# Autodesk Inventor assembly: CL5-100
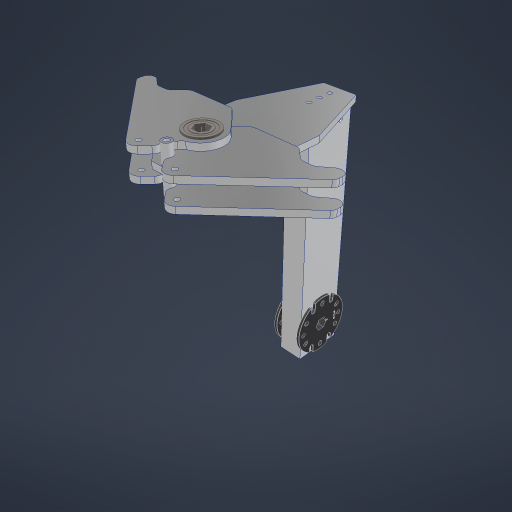
[picture p0: Inventor's stored thumbnail of the model, 512x512]
Saved by Autodesk Inventor 2023.4 (Build 274418000, 418)
## iProperties
Created: 2025-02-04
Part Number: CL5-100
Document SubType Name: Assembly
Designer: brand
Author: brand
## Documents named in this file (10)
- C:\Users\brand\OneDrive\Documents\GitHub\robotics 23\2025-ReefScape---CAD\Climber\CL5\CL5-100.iam
- C:\Users\brand\OneDrive\Documents\GitHub\robotics 23\2025-ReefScape---CAD\Field Items\Full Field\FE-2025\GE-25201.iam
- C:\Users\brand\OneDrive\Documents\GitHub\robotics 23\2025-ReefScape---CAD\Climber\CL4\02_Barb Assembly (1)\02_Barb Assembly (1).iam
- C:\Users\brand\OneDrive\Documents\GitHub\robotics 23\2025-ReefScape---CAD\COMMON PARTS\HUBS\WCP-1388.ipt
- C:\Users\brand\OneDrive\Documents\GitHub\robotics 23\2025-ReefScape---CAD\Climber\CL5\CL5-001.ipt
- C:\Users\brand\OneDrive\Documents\GitHub\robotics 23\2025-ReefScape---CAD\Elevator\EL2\EL2-005.ipt
- C:\Users\brand\OneDrive\Documents\GitHub\robotics 23\2025-ReefScape---CAD\Climber\CL5\CL5-002.ipt
- C:\Users\brand\OneDrive\Documents\GitHub\robotics 23\2025-ReefScape---CAD\Climber\CL5\CL5-003.ipt
- C:\Users\brand\OneDrive\Documents\GitHub\robotics 23\2025-ReefScape---CAD\Climber\CL5\CL5-004.ipt
- C:\Users\brand\OneDrive\Documents\GitHub\robotics 23\2025-ReefScape---CAD\COMMON PARTS\BEARINGS\0_500_Hex_ID_x_1_125_OD_x_0_313_WD_Flanged_Bearing_v2_217-3875.ipt
## Components (18 placed, 9 different names)
1. CL5-001:1 — Mate:7, Flush:6, Flush:7, Insert:2, Mate:14, Insert:3, Mate:15, Mate:16, Flush:9, Insert:11, Insert:12
2. GE-25201:1 [sub-assembly] — Mate:7
3. 02_Barb Assembly (1):1 [sub-assembly] — Flush:6, Flush:7
4. WCP-1388:1 — Insert:2, Mate:14
5. WCP-1388:2 — Insert:3, Mate:15
6. EL2-005:1 — Insert:11, Insert:12, Insert:13, Insert:14
7. CL5-002:1 — Mate:18, Mate:19, Mate:20, Mate:21, Flush:9, Insert:4, Insert:5, Insert:8, Insert:13, Insert:14
8. CL5-003:1 — Mate:18, Insert:9, Mate:26
9. CL5-004:1 — Insert:4, Mate:28, Mate:29
10. CL5-003:2 — Mate:21, Insert:7, Mate:28
11. CL5-003:4 — Mate:19, Insert:6, Mate:29
12. CL5-003:5 — Mate:20, Insert:10, Mate:27
13. CL5-004:2 — Insert:5, Mate:26, Mate:27
14. 0_500_Hex_ID_x_1_125_OD_x_0_313_WD_Flanged_Bearing_v2_217-3875:1 — Insert:8, Mate:22, Mate:24
15. 0_500_Hex_ID_x_1_125_OD_x_0_313_WD_Flanged_Bearing_v2_217-3875:2 — Insert:10, Mate:25
16. 0_500_Hex_ID_x_1_125_OD_x_0_313_WD_Flanged_Bearing_v2_217-3875:3 — Insert:9, Mate:24, Mate:25
17. 0_500_Hex_ID_x_1_125_OD_x_0_313_WD_Flanged_Bearing_v2_217-3875:4 — Insert:7, Mate:22, Mate:23
18. 0_500_Hex_ID_x_1_125_OD_x_0_313_WD_Flanged_Bearing_v2_217-3875:5 — Insert:6, Mate:23
## Relationships (32: Mate 16, Insert 13, Flush 3)
- Mate:7: CL5-001:1 ↔ GE-25201:1
- Flush:6: CL5-001:1 ↔ 02_Barb Assembly (1):1
- Flush:7: CL5-001:1 ↔ 02_Barb Assembly (1):1
- Insert:2: CL5-001:1 ↔ WCP-1388:1
- Mate:14: CL5-001:1 ↔ WCP-1388:1
- Insert:3: CL5-001:1 ↔ WCP-1388:2
- Mate:15: CL5-001:1 ↔ WCP-1388:2
- Mate:16: CL5-001:1
- Mate:18: CL5-002:1 ↔ CL5-003:1
- Mate:19: CL5-002:1 ↔ CL5-003:4
- Mate:20: CL5-002:1 ↔ CL5-003:5
- Mate:21: CL5-002:1 ↔ CL5-003:2
- Flush:9: CL5-001:1 ↔ CL5-002:1
- Insert:4: CL5-002:1 ↔ CL5-004:1
- Insert:5: CL5-002:1 ↔ CL5-004:2
- Insert:6: CL5-003:4 ↔ 0_500_Hex_ID_x_1_125_OD_x_0_313_WD_Flanged_Bearing_v2_217-3875:5
- Insert:7: CL5-003:2 ↔ 0_500_Hex_ID_x_1_125_OD_x_0_313_WD_Flanged_Bearing_v2_217-3875:4
- Insert:8: CL5-002:1 ↔ 0_500_Hex_ID_x_1_125_OD_x_0_313_WD_Flanged_Bearing_v2_217-3875:1
- Insert:9: CL5-003:1 ↔ 0_500_Hex_ID_x_1_125_OD_x_0_313_WD_Flanged_Bearing_v2_217-3875:3
- Insert:10: CL5-003:5 ↔ 0_500_Hex_ID_x_1_125_OD_x_0_313_WD_Flanged_Bearing_v2_217-3875:2
- Mate:22: 0_500_Hex_ID_x_1_125_OD_x_0_313_WD_Flanged_Bearing_v2_217-3875:1 ↔ 0_500_Hex_ID_x_1_125_OD_x_0_313_WD_Flanged_Bearing_v2_217-3875:4
- Mate:23: 0_500_Hex_ID_x_1_125_OD_x_0_313_WD_Flanged_Bearing_v2_217-3875:4 ↔ 0_500_Hex_ID_x_1_125_OD_x_0_313_WD_Flanged_Bearing_v2_217-3875:5
- Mate:24: 0_500_Hex_ID_x_1_125_OD_x_0_313_WD_Flanged_Bearing_v2_217-3875:1 ↔ 0_500_Hex_ID_x_1_125_OD_x_0_313_WD_Flanged_Bearing_v2_217-3875:3
- Mate:25: 0_500_Hex_ID_x_1_125_OD_x_0_313_WD_Flanged_Bearing_v2_217-3875:2 ↔ 0_500_Hex_ID_x_1_125_OD_x_0_313_WD_Flanged_Bearing_v2_217-3875:3
- Mate:26: CL5-003:1 ↔ CL5-004:2
- Mate:27: CL5-003:5 ↔ CL5-004:2
- Mate:28: CL5-004:1 ↔ CL5-003:2
- Mate:29: CL5-004:1 ↔ CL5-003:4
- Insert:11: CL5-001:1 ↔ EL2-005:1
- Insert:12: CL5-001:1 ↔ EL2-005:1
- Insert:13: EL2-005:1 ↔ CL5-002:1
- Insert:14: EL2-005:1 ↔ CL5-002:1
